# Autodesk Inventor assembly: flex_wheel
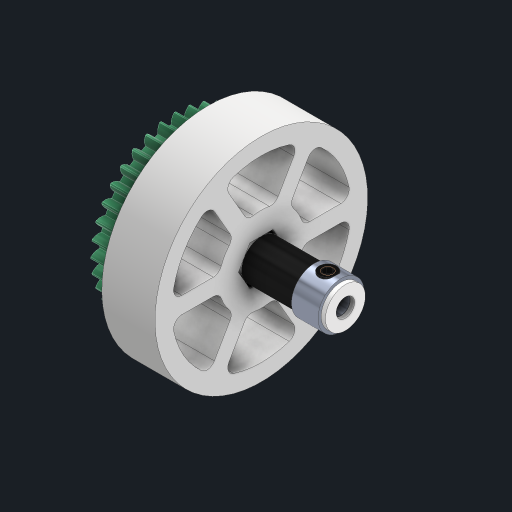
[picture p0: Inventor's stored thumbnail of the model, 512x512]
Saved by Autodesk Inventor 2024 (Build 280153000, 153)
## iProperties
Created: 2023-08-17
Part Number: flex_wheel
Document SubType Name: Assembly
Designer: avere
Author: avere
## Documents named in this file (11)
- D:\vex_robotics\hardware\cad\scrap_v0.1\chassis\flex_wheel.iam
- D:\vex_robotics\hardware\cad\VEX-CAD-Inventor-1.41\Motion\Gears\LS 36T Gear.ipt
- D:\vex_robotics\hardware\cad\VEX-CAD-Inventor-1.41\Motion\Spacers\Spacer Nylon .375 OD\NSpacer .375 OD x .500.ipt
- D:\vex_robotics\hardware\cad\VEX-CAD-Inventor-1.41\Motion\Spacers\Spacer Nylon .375 OD.ipt
- D:\vex_robotics\hardware\cad\VEX-CAD-Inventor-1.41\Motion\Shaft LS\Shaft Collar ipts\Shaft Collar Set Screw.ipt
- D:\vex_robotics\hardware\cad\VEX-CAD-Inventor-1.41\Motion\Spacers\Washer Teflon\TWasher .375 OD x .04000.ipt
- D:\vex_robotics\hardware\cad\VEX-CAD-Inventor-1.41\Motion\Spacers\Washer Teflon.ipt
- D:\vex_robotics\hardware\cad\VEX-CAD-Inventor-1.41\Motion\Spacers\Washer Steel\SWasher .375 OD x .015625.ipt
- D:\vex_robotics\hardware\cad\VEX-CAD-Inventor-1.41\Motion\Spacers\Washer Steel.ipt
- D:\vex_robotics\hardware\cad\VEX-CAD-Inventor-1.41\Motion\Wheels\Flex Wheels\2.000 Flex Wheel\2.000 30A .500.ipt
- D:\vex_robotics\hardware\cad\VEX-CAD-Inventor-1.41\Motion\Wheels\Flex Wheels\2.000 Flex Wheel.ipt
## Components (6 placed, 6 different names)
1. LS 36T Gear:1 — Insert:6
2. NSpacer .375 OD x .500:2 — Insert:7
3. Shaft Collar Set Screw:1
4. TWasher .375 OD x .04000:1
5. SWasher .375 OD x .015625:1
6. 2.000 30A .500:1 — Insert:6, Insert:7
## Relationships (5: Insert 5)
- [Insert]: NSpacer .375 OD x .500:2 ↔ Shaft Collar Set Screw:1
- [Insert]: LS 36T Gear:1 ↔ SWasher .375 OD x .015625:1
- [Insert]: Shaft Collar Set Screw:1 ↔ TWasher .375 OD x .04000:1
- Insert:6: LS 36T Gear:1 ↔ 2.000 30A .500:1
- Insert:7: NSpacer .375 OD x .500:2 ↔ 2.000 30A .500:1
